# Autodesk Inventor assembly: Shield
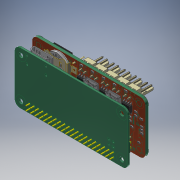
[picture p0: Inventor's stored thumbnail of the model, 180x180]
Saved by Autodesk Inventor 2017 (Build 210142000, 142)
## iProperties
Created: 2017-09-23
Part Number: Shield
Document SubType Name: Assembly
Designer: P. Baesso
Author: P. Baesso
## iProperties of the stored document _C-95-01-20-D-TE.ipt
Created: 2017-09-23
Part Number: _C-95-01-20-D-TE
Material: Generic
Document SubType Name: Modeling
Designer: P. Baesso
Density: 1 g/cm^3
Appearance: Default
Author: P. Baesso
Revision Number: NONE
## iProperties of the stored document BCS-120-F-D-TE.iam
Created: 2017-09-21
Part Number: BCS-120-F-D-TE
Description: STEP AP214
Document SubType Name: Assembly
Designer: P. Baesso
Sending System: PARTsolutions
Title: p:/temp/worker_11/5296_5584/app_90_02017092119583060957461192d056f_000000_00_00_000000/format_0/BCS-120-F-D-TE.stp
Revision Number: NONE
## iProperties of the stored document _BCS-120-D-TE_socket.ipt
Created: 2017-09-23
Part Number: _BCS-120-D-TE_socket
Material: Generic
Document SubType Name: Modeling
Designer: P. Baesso
Density: 1 g/cm^3
Appearance: Default
Author: P. Baesso
Revision Number: NONE
## Documents named in this file (8)
- **C:\Rymapt\ethoscope_hardware\Shield\Shield.iam*LocalDocs*xNv4zsbinXgbgedo4Y400ht4x0a*_C-95-01-20-D-TE.ipt
- **C:\Rymapt\ethoscope_hardware\Shield\Shield.iam*LocalDocs*x2kthyjz3Ke0xe2cx2asym0h5Sh*BCS-120-F-D-TE.iam
- **C:\Rymapt\ethoscope_hardware\Shield\Shield.iam*LocalDocs*xRi1hqhs0TgazeqcsRydyaihtIe*_BCS-120-D-TE_socket.ipt
- C:\Rymapt\ethoscope_hardware\Shield\Shield.iam
- C:\Rymapt\ethoscope_hardware\PiZero\RapberryPiZero.iam
- C:\Rymapt\ethoscope_hardware\Shield\Files\User Library-CR1225.iam
- C:\Rymapt\ethoscope_hardware\Shield\Files\PCB_R2D2.iam
- P:\cad\steps_files\BCS-120-F-D-TE.stp
## Components (4 placed, 4 different names)
1. RapberryPiZero:1 [sub-assembly] — Angle:1, Mate:1, Mate:2, Mate:3, Flush:2, Flush:3
2. BCS-120-F-D-TE:1 [sub-assembly] — Angle:1, Mate:1, Mate:2, Mate:3, Flush:1
3. User Library-CR1225:1 [sub-assembly] — Flush:4, Tangent:1, Tangent:2
4. PCB_R2D2:1 [sub-assembly] — Flush:1, Flush:2, Flush:3, Flush:4, Tangent:1, Tangent:2
## Relationships (10: Flush 4, Mate 3, Tangent 2, Angle 1)
- Angle:1 (0 deg): RapberryPiZero:1 ↔ BCS-120-F-D-TE:1
- Mate:1 (0.1 mm): RapberryPiZero:1 ↔ BCS-120-F-D-TE:1
- Mate:2 (-0.15 mm): RapberryPiZero:1 ↔ BCS-120-F-D-TE:1
- Mate:3 (-0.254 mm): RapberryPiZero:1 ↔ BCS-120-F-D-TE:1
- Flush:1 (-1.6 mm): BCS-120-F-D-TE:1 ↔ PCB_R2D2:1
- Flush:2: RapberryPiZero:1 ↔ PCB_R2D2:1
- Flush:3: RapberryPiZero:1 ↔ PCB_R2D2:1
- Flush:4 (0.1 mm): User Library-CR1225:1 ↔ PCB_R2D2:1
- Tangent:1 (0.1 mm): User Library-CR1225:1 ↔ PCB_R2D2:1
- Tangent:2 (0.15 mm): User Library-CR1225:1 ↔ PCB_R2D2:1
